# Autodesk Inventor assembly: Bancada de Lavagem Mãos - 1150 x 370 x 900h
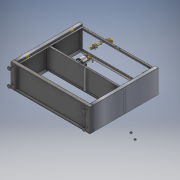
[picture p0: Inventor's stored thumbnail of the model, 180x180]
Saved by Autodesk Inventor 2017 (Build 210142000, 142)
## iProperties
Created: 2019-06-15
Part Number: Bancada de Lavagem Mãos - 1150 x 370 x 900h
Document SubType Name: Assembly
Designer: leonardo.prado
Mass: 36378 g
Surface Area: 63880.5 cm^2
Volume: 11799.5 cm^3
Author: leonardo.prado
## Documents named in this file (29)
- D:\LEONARDO\Desktop\3 - Inventor\Moveis em Aço Inox\MTC-2319 - Influenza\7.2 - Bancada de Lavagem de Mãos\Montagens\Bancada de Lavagem Mãos - 1150 x 370 x 900h.iam
- D:\LEONARDO\Desktop\3 - Inventor\Moveis em Aço Inox\MTC-2319 - Influenza\7.2 - Bancada de Lavagem de Mãos\Componentes\Bancada Lavagem de Mãos.ipt
- D:\LEONARDO\Desktop\3 - Inventor\Moveis em Aço Inox\MTC-2319 - Influenza\1 - Acessórios\Torneiras\Deca\Lux 1180 C\Componentes\DecaLux - 1180.C.ipt
- D:\LEONARDO\Desktop\3 - Inventor\Moveis em Aço Inox\MTC-2319 - Influenza\1 - Acessórios\Valvulas Escoamento\1. 1.2 - Deca 1623.ipt
- D:\LEONARDO\Desktop\3 - Inventor\Moveis em Aço Inox\MTC-2319 - Influenza\7.2 - Bancada de Lavagem de Mãos\Componentes\Base.ipt
- D:\LEONARDO\Desktop\3 - Inventor\Moveis em Aço Inox\MTC-2319 - Influenza\7.2 - Bancada de Lavagem de Mãos\Componentes\Lateral -A.ipt
- D:\LEONARDO\Desktop\3 - Inventor\Moveis em Aço Inox\MTC-2319 - Influenza\7.2 - Bancada de Lavagem de Mãos\Componentes\Lateral -A1.ipt
- D:\LEONARDO\Desktop\3 - Inventor\Moveis em Aço Inox\MTC-2319 - Influenza\7.2 - Bancada de Lavagem de Mãos\Componentes\Prateleira.ipt
- D:\LEONARDO\Desktop\3 - Inventor\Moveis em Aço Inox\MTC-2319 - Influenza\1 - Acessórios\Sifões\Montagens\Sifão.iam
- D:\LEONARDO\Desktop\3 - Inventor\Moveis em Aço Inox\MTC-2319 - Influenza\7.2 - Bancada de Lavagem de Mãos\Componentes\Chapa Fixação Pé Nivelador.ipt
- D:\LEONARDO\Desktop\3 - Inventor\Moveis em Aço Inox\MTC-2319 - Influenza\1 - Acessórios\Sapatas Niveladora\Componentes\Sapata Niveladora.ipt
- D:\MTC\Documents\Inventor\Content Center Files\R2017\en-US\AS 1112 (4)\AS 1112 - M10(2).ipt
- D:\LEONARDO\Desktop\3 - Inventor\Moveis em Aço Inox\MTC-2319 - Influenza\7.2 - Bancada de Lavagem de Mãos\Componentes\Chapa Fixação Pé Nivelador1.ipt
- D:\LEONARDO\Desktop\3 - Inventor\Moveis em Aço Inox\MTC-2319 - Influenza\1 - Acessórios\Sapatas Niveladora\Componentes\Sapata Niveladora1.ipt
- D:\LEONARDO\Desktop\3 - Inventor\Moveis em Aço Inox\MTC-2319 - Influenza\7.2 - Bancada de Lavagem de Mãos\Componentes\Porta.ipt
- D:\LEONARDO\Desktop\3 - Inventor\Moveis em Aço Inox\MTC-2319 - Influenza\1 - Acessórios\Dobradiças\Montagens\DB-38mm.iam
- D:\LEONARDO\Desktop\3 - Inventor\Moveis em Aço Inox\MTC-2319 - Influenza\1 - Acessórios\Puxadores\Puxador 110x40mm.ipt
- D:\MTC\Documents\Inventor\Content Center Files\R2017\en-US\AS 1427(04)\AS 1427 - M4 x 12(5) I.ipt
- D:\LEONARDO\Desktop\3 - Inventor\Moveis em Aço Inox\MTC-2319 - Influenza\7.2 - Bancada de Lavagem de Mãos\Componentes\Porta1.ipt
- D:\LEONARDO\Desktop\3 - Inventor\Moveis em Aço Inox\MTC-2319 - Influenza\1 - Acessórios\Dobradiças\Montagens\DB-38mm2.iam
- D:\LEONARDO\Desktop\3 - Inventor\Moveis em Aço Inox\MTC-2319 - Influenza\1 - Acessórios\Puxadores\Puxador 110x40mm1.ipt
- D:\MTC\Documents\Inventor\Content Center Files\R2017\en-US\DIN 125-1  A\DIN 125 - A 8,4.ipt
- D:\MTC\Documents\Inventor\Content Center Files\R2017\en-US\AS 1110\AS 1110 - M8 x 20.ipt
- D:\LEONARDO\Desktop\3 - Inventor\Moveis em Aço Inox\MTC-2319 - Influenza\7.2 - Bancada de Lavagem de Mãos\Componentes\Reforço Bandeja Prateleira.ipt
- D:\LEONARDO\Desktop\3 - Inventor\Moveis em Aço Inox\MTC-2319 - Influenza\1 - Acessórios\Imã Permanente\Componentes\Imã 22mm.ipt
- D:\LEONARDO\Desktop\3 - Inventor\Moveis em Aço Inox\MTC-2319 - Influenza\7.2 - Bancada de Lavagem de Mãos\Componentes\Perfil L 30 x 20.ipt
- D:\LEONARDO\Desktop\3 - Inventor\Moveis em Aço Inox\MTC-2319 - Influenza\7.2 - Bancada de Lavagem de Mãos\Componentes\Perfil J 25x25x10 - 930.ipt
- D:\LEONARDO\Desktop\3 - Inventor\Moveis em Aço Inox\MTC-2319 - Influenza\7.2 - Bancada de Lavagem de Mãos\Componentes\Batente batoque Inferior.ipt
- D:\LEONARDO\Desktop\3 - Inventor\Moveis em Aço Inox\MTC-2319 - Influenza\1 - Acessórios\Imã Permanente\Componentes\Atrack 60 x 20 x 10.ipt
## Components (47 placed, 28 different names)
1. Bancada Lavagem de Mãos:1 — Flush:1, Flush:2, Flush:3, Mate:21, Mate:22, Mate:23, Mate:24, Flush:4, Flush:5
2. DecaLux - 1180.C:1 — Mate:21, Mate:22
3. 1. 1.2 - Deca 1623:1 — Mate:23, Mate:24, Mate:28
4. Base:2 — Mate:25, Flush:4, Flush:5, Flush:6, Flush:7, Mate:29, Mate:30, Mate:31, Flush:8, Mate:40, Flush:9, Mate:41, Flush:10, Flush:11, Mate:66, Mate:72
5. Lateral -A:1 — Flush:6, Mate:43, Mate:44, Insert:5, Insert:6, Mate:61, Flush:16, Mate:67, Mate:69, Mate:70
6. Lateral -A1:1 — Mate:41, Flush:10, Flush:11, Mate:42, Insert:7, Insert:8, Mate:68, Flush:17, Flush:18, Flush:19
7. Prateleira:1 — Flush:7, Mate:43, Mate:44, Mate:59, Mate:60
8. Sifão:1 [sub-assembly] — Mate:28
9. Chapa Fixação Pé Nivelador:1 — Mate:29, Mate:30, Mate:31, Mate:33, Mate:35, Insert:1, Insert:2
10. Sapata Niveladora:1 — Mate:32, Mate:33
11. Sapata Niveladora:2 — Mate:34, Mate:35
12. AS 1112 (4) - Metric M10:1 — Insert:1
13. AS 1112 (4) - Metric M10:2 — Insert:2
14. Chapa Fixação Pé Nivelador1:1 — Mate:36, Mate:38, Insert:3, Insert:4
15. Sapata Niveladora1:1 — Mate:36, Mate:37
16. Sapata Niveladora1:2 — Mate:38, Mate:39
17. AS 1112 (4) - Metric M10:3 — Insert:3
18. AS 1112 (4) - Metric M10:4 — Insert:4
19. Porta:1 — Flush:8, Mate:40, Flush:9, Mate:42, Mate:45, Flush:12, Flush:13, Mate:46, Mate:47, Mate:48, Mate:49, Mate:50
20. Puxador 110x40mm:1 — Mate:46, Mate:47, Mate:48
21. AS 1427 H - Metric M4 x 12:1 — Mate:49
22. AS 1427 H - Metric M4 x 12:2 — Mate:50
23. Porta1:1 — Flush:14, Flush:15, Mate:51, Mate:52, Mate:53, Mate:54, Mate:55, Mate:56, Mate:66, Flush:16, Mate:67
24. Puxador 110x40mm1:1 — Mate:52, Mate:53, Mate:54
25. AS 1427 H - Metric M4 x 12:3 — Mate:55
26. AS 1427 H - Metric M4 x 12:4 — Mate:56
27. DIN 125-1 A A 8,4:1 — Insert:5, Insert:12
28. DIN 125-1 A A 8,4:2 — Insert:6, Insert:11
29. DIN 125-1 A A 8,4:3 — Insert:7, Insert:9
30. DIN 125-1 A A 8,4:4 — Insert:8, Insert:10
31. AS 1110 - Metric M8 x 20:1 — Insert:9
32. AS 1110 - Metric M8 x 20:2 — Insert:10
33. AS 1110 - Metric M8 x 20:3 — Insert:11
34. AS 1110 - Metric M8 x 20:4 — Insert:12
35. Reforço Bandeja Prateleira:1 — Mate:59, Mate:60, Mate:61
36. Imã 22mm:1
37. Imã 22mm:2
38. Batente Superior Gabinete:1 — Mate:68, Flush:17, Flush:18, Mate:76, Mate:77
39. Perfil J 25x25x10 - 930:1 — Mate:69, Mate:70, Mate:71
40. Batente batoque Inferior:1 — Mate:72, Flush:19, Mate:73, Mate:74, Mate:75
41. AS 1427 H - Metric M4 x 12:5 — Mate:74
42. AS 1427 H - Metric M4 x 12:6 — Mate:75
43. Atrack 60 x 20 x 10:1 — Mate:76, Mate:77, Flush:20
44. DB-38mm:1 [sub-assembly] — Mate:45, Flush:12, Flush:13
45. DB-38mm:2 [sub-assembly]
46. DB-38mm2:1 [sub-assembly] — Flush:14, Flush:15, Mate:51
47. DB-38mm2:2 [sub-assembly]
## Component patterns: (2 elements, first: DB-38mm:1), (2 elements, first: DB-38mm2:1)
## Relationships (81: Mate 49, Flush 20, Insert 12)
- Flush:1 (-900 mm): Bancada Lavagem de Mãos:1
- Flush:2: Bancada Lavagem de Mãos:1
- Flush:3: Bancada Lavagem de Mãos:1
- Mate:21: Bancada Lavagem de Mãos:1 ↔ DecaLux - 1180.C:1
- Mate:22: Bancada Lavagem de Mãos:1 ↔ DecaLux - 1180.C:1
- Mate:23: Bancada Lavagem de Mãos:1 ↔ 1. 1.2 - Deca 1623:1
- Mate:24: Bancada Lavagem de Mãos:1 ↔ 1. 1.2 - Deca 1623:1
- Mate:25 (50 mm): Base:2
- Flush:4: Bancada Lavagem de Mãos:1 ↔ Base:2
- Flush:5: Bancada Lavagem de Mãos:1 ↔ Base:2
- Flush:6: Base:2 ↔ Lateral -A:1
- Flush:7 (-385 mm): Base:2 ↔ Prateleira:1
- Mate:28: 1. 1.2 - Deca 1623:1 ↔ Sifão:1
- Mate:29: Base:2 ↔ Chapa Fixação Pé Nivelador:1
- Mate:30: Base:2 ↔ Chapa Fixação Pé Nivelador:1
- Mate:31: Base:2 ↔ Chapa Fixação Pé Nivelador:1
- Mate:32: Sapata Niveladora:1
- Mate:33: Chapa Fixação Pé Nivelador:1 ↔ Sapata Niveladora:1
- Mate:34: Sapata Niveladora:2
- Mate:35: Chapa Fixação Pé Nivelador:1 ↔ Sapata Niveladora:2
- Insert:1: Chapa Fixação Pé Nivelador:1 ↔ AS 1112 (4) - Metric M10:1
- Insert:2: Chapa Fixação Pé Nivelador:1 ↔ AS 1112 (4) - Metric M10:2
- Mate:36: Chapa Fixação Pé Nivelador1:1 ↔ Sapata Niveladora1:1
- Mate:37: Sapata Niveladora1:1
- Mate:38: Chapa Fixação Pé Nivelador1:1 ↔ Sapata Niveladora1:2
- Mate:39: Sapata Niveladora1:2
- Insert:3: Chapa Fixação Pé Nivelador1:1 ↔ AS 1112 (4) - Metric M10:3
- Insert:4: Chapa Fixação Pé Nivelador1:1 ↔ AS 1112 (4) - Metric M10:4
- Flush:8: Base:2 ↔ Porta:1
- Mate:40 (2 mm): Base:2 ↔ Porta:1
- Flush:9: Base:2 ↔ Porta:1
- Mate:41: Base:2 ↔ Lateral -A1:1
- Flush:10: Base:2 ↔ Lateral -A1:1
- Flush:11: Base:2 ↔ Lateral -A1:1
- Mate:42 (4 mm): Lateral -A1:1 ↔ Porta:1
- Mate:43: Lateral -A:1 ↔ Prateleira:1
- Mate:44: Lateral -A:1 ↔ Prateleira:1
- Mate:45: Porta:1 ↔ DB-38mm:1
- Flush:12 (100 mm): Porta:1 ↔ DB-38mm:1
- Flush:13 (-13.5 mm): Porta:1 ↔ DB-38mm:1
- Mate:46: Porta:1 ↔ Puxador 110x40mm:1
- Mate:47: Porta:1 ↔ Puxador 110x40mm:1
- Mate:48: Porta:1 ↔ Puxador 110x40mm:1
- Mate:49: Porta:1 ↔ AS 1427 H - Metric M4 x 12:1
- Mate:50: Porta:1 ↔ AS 1427 H - Metric M4 x 12:2
- Flush:14 (-13.5 mm): Porta1:1 ↔ DB-38mm2:1
- Flush:15 (100 mm): Porta1:1 ↔ DB-38mm2:1
- Mate:51: Porta1:1 ↔ DB-38mm2:1
- Mate:52: Porta1:1 ↔ Puxador 110x40mm1:1
- Mate:53: Porta1:1 ↔ Puxador 110x40mm1:1
- Mate:54: Porta1:1 ↔ Puxador 110x40mm1:1
- Mate:55: Porta1:1 ↔ AS 1427 H - Metric M4 x 12:3
- Mate:56: Porta1:1 ↔ AS 1427 H - Metric M4 x 12:4
- Insert:5: Lateral -A:1 ↔ DIN 125-1 A A 8,4:1
- Insert:6: Lateral -A:1 ↔ DIN 125-1 A A 8,4:2
- Insert:7: Lateral -A1:1 ↔ DIN 125-1 A A 8,4:3
- Insert:8: Lateral -A1:1 ↔ DIN 125-1 A A 8,4:4
- Insert:9: DIN 125-1 A A 8,4:3 ↔ AS 1110 - Metric M8 x 20:1
- Insert:10: DIN 125-1 A A 8,4:4 ↔ AS 1110 - Metric M8 x 20:2
- Insert:11: DIN 125-1 A A 8,4:2 ↔ AS 1110 - Metric M8 x 20:3
- Insert:12: DIN 125-1 A A 8,4:1 ↔ AS 1110 - Metric M8 x 20:4
- Mate:59: Prateleira:1 ↔ Reforço Bandeja Prateleira:1
- Mate:60: Prateleira:1 ↔ Reforço Bandeja Prateleira:1
- Mate:61 (450.3 mm): Lateral -A:1 ↔ Reforço Bandeja Prateleira:1
- Mate:66 (2 mm): Base:2 ↔ Porta1:1
- Flush:16: Lateral -A:1 ↔ Porta1:1
- Mate:67 (4 mm): Lateral -A:1 ↔ Porta1:1
- Mate:68: Lateral -A1:1 ↔ Batente Superior Gabinete:1
- Flush:17: Lateral -A1:1 ↔ Batente Superior Gabinete:1
- Flush:18: Lateral -A1:1 ↔ Batente Superior Gabinete:1
- Mate:69: Lateral -A:1 ↔ Perfil J 25x25x10 - 930:1
- Mate:70: Lateral -A:1 ↔ Perfil J 25x25x10 - 930:1
- Mate:71: Perfil J 25x25x10 - 930:1
- Mate:72: Base:2 ↔ Batente batoque Inferior:1
- Flush:19: Lateral -A1:1 ↔ Batente batoque Inferior:1
- Mate:73: Batente batoque Inferior:1
- Mate:74: Batente batoque Inferior:1 ↔ AS 1427 H - Metric M4 x 12:5
- Mate:75: Batente batoque Inferior:1 ↔ AS 1427 H - Metric M4 x 12:6
- Mate:76: Batente Superior Gabinete:1 ↔ Atrack 60 x 20 x 10:1
- Mate:77: Batente Superior Gabinete:1 ↔ Atrack 60 x 20 x 10:1
- Flush:20: Atrack 60 x 20 x 10:1
